# Autodesk Inventor assembly: Ecnlosure01
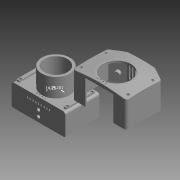
[picture p0: Inventor's stored thumbnail of the model, 180x180]
Saved by Autodesk Inventor 2013 (Build 170138000, 138)
## iProperties
Created: 2014-04-13
Part Number: Ecnlosure01
Document SubType Name: Assembly
Designer: spichelh
Author: spichelh
## Documents named in this file (12)
- C:\Users\spichelh\Documents\GitHub\beta-hardware\Enclosure\Version 002\Enclosure01.iam
- C:\Users\spichelh\Documents\GitHub\beta-hardware\Enclosure\Version 002\Enclosure01.ipt
- C:\Users\spichelh\Documents\GitHub\beta-hardware\Enclosure\Version 002\PCB01.ipt
- C:\Users\spichelh\Documents\GitHub\beta-hardware\Enclosure\Version 002\Microzed01.ipt
- C:\Users\spichelh\Documents\GitHub\beta-hardware\Enclosure\Version 002\AddonPCB01.ipt
- C:\Users\spichelh\Documents\GitHub\beta-hardware\Enclosure\Version 002\Enclosure-Backplate01.ipt
- C:\Users\spichelh\Documents\GitHub\beta-hardware\Enclosure\Version 002\Nikon Mount.ipt
- C:\Users\spichelh\Documents\GitHub\beta-hardware\Enclosure\Version 002\KAC12040.ipt
- C:\Users\spichelh\Documents\GitHub\beta-hardware\Enclosure\Version 002\IRGlass.ipt
- C:\Users\spichelh\Documents\GitHub\beta-hardware\Enclosure\Version 002\Nikon Base.ipt
- C:\Users\spichelh\Documents\GitHub\beta-hardware\Enclosure\Version 002\Cooler.ipt
- C:\Users\spichelh\Documents\GitHub\beta-hardware\Enclosure\Version 002\Enclosure02.ipt
## Components (11 placed, 11 different names)
1. Nikon Base:1 — Mate:8, Mate:11, Mate:16, Mate:17, Flush:10, Flush:11, Flush:12, Mate:18, Mate:19, Mate:23, Mate:24, Mate:25, Flush:13, Flush:14, Flush:15
2. PCB01:1 — Mate:1, Flush:1, Flush:2, Mate:23, Mate:24
3. Microzed01:1 — Mate:1, Flush:1, Flush:2, Flush:3, Mate:2, Flush:4
4. AddonPCB01:1 — Flush:3, Mate:2, Flush:4
5. Nikon Mount:1 — Mate:8, Mate:11, Mate:17, Mate:20, Mate:21, Mate:22, Mate:26
6. Enclosure01:1 — Mate:25, Flush:13, Mate:26, Flush:14, Flush:16, Flush:17, Flush:18, Mate:27
7. Enclosure-Backplate01:1 — Flush:18, Mate:27
8. KAC12040:1 — Mate:16, Mate:18, Mate:19
9. IRGlass:1 — Mate:20, Mate:21, Mate:22
10. Cooler:1 — Flush:15, Flush:16, Flush:17
11. Enclosure02:1
## Relationships (29: Mate 16, Flush 13)
- Mate:1 (5 mm): PCB01:1 ↔ Microzed01:1
- Flush:1: PCB01:1 ↔ Microzed01:1
- Flush:2: PCB01:1 ↔ Microzed01:1
- Flush:3: Microzed01:1 ↔ AddonPCB01:1
- Mate:2 (10 mm): Microzed01:1 ↔ AddonPCB01:1
- Flush:4: Microzed01:1 ↔ AddonPCB01:1
- Mate:8: Nikon Base:1 ↔ Nikon Mount:1
- Mate:11: Nikon Base:1 ↔ Nikon Mount:1
- Mate:16: Nikon Base:1 ↔ KAC12040:1
- Mate:17: Nikon Base:1 ↔ Nikon Mount:1
- Flush:10: Nikon Base:1
- Flush:11: Nikon Base:1
- Flush:12: Nikon Base:1
- Mate:18 (4 mm): Nikon Base:1 ↔ KAC12040:1
- Mate:19 (10.7 mm): Nikon Base:1 ↔ KAC12040:1
- Mate:20: Nikon Mount:1 ↔ IRGlass:1
- Mate:21 (0.5 mm): Nikon Mount:1 ↔ IRGlass:1
- Mate:22 (0.5 mm): Nikon Mount:1 ↔ IRGlass:1
- Mate:23: Nikon Base:1 ↔ PCB01:1
- Mate:24: Nikon Base:1 ↔ PCB01:1
- Mate:25: Nikon Base:1 ↔ Enclosure01:1
- Flush:13: Nikon Base:1 ↔ Enclosure01:1
- Mate:26: Nikon Mount:1 ↔ Enclosure01:1
- Flush:14: Nikon Base:1 ↔ Enclosure01:1
- Flush:15: Nikon Base:1 ↔ Cooler:1
- Flush:16: Enclosure01:1 ↔ Cooler:1
- Flush:17 (33 mm): Enclosure01:1 ↔ Cooler:1
- Flush:18: Enclosure01:1 ↔ Enclosure-Backplate01:1
- Mate:27: Enclosure01:1 ↔ Enclosure-Backplate01:1
